# Autodesk Inventor assembly: szafka
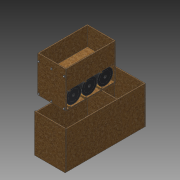
[picture p0: Inventor's stored thumbnail of the model, 180x180]
Saved by Autodesk Inventor 2013 (Build 170138000, 138)
## iProperties
Created: 2014-04-26
Part Number: szafka
Document SubType Name: Assembly
Designer: Masta
Author: Masta
## Documents named in this file (8)
- D:\prusa i3\assembly\szafka\szafka.iam
- D:\prusa i3\assembly\szafka\bok.ipt
- D:\prusa i3\assembly\szafka\tyl.ipt
- D:\prusa i3\assembly\szafka\podstawa.ipt
- D:\prusa i3\assembly\szafka\polka.ipt
- D:\prusa i3\assembly\szafka\rolka_filamentu.ipt
- D:\prusa i3\assembly\szafka\gora.ipt
- D:\prusa i3\assembly\szafka\wozek.iam
## Components (22 placed, 7 different names)
1. bok:1 — Flush:2, Flush:5, Mate:5, Flush:7, Mate:10, Flush:9, Mate:13
2. bok:2 — Flush:8, Mate:6, Mate:7
3. tyl:1 — Mate:1, Flush:2, Mate:4, Flush:6, Mate:5, Flush:7, Flush:8, Mate:6, Mate:9, Mate:11, Flush:10, Mate:14
4. podstawa:1 — Mate:4, Flush:5, Flush:6, Mate:7, Mate:12
5. polka:1 — Mate:9, Mate:10, Mate:15
6. gora:1 — Mate:11, Flush:9, Flush:10, Mate:15
7. wozek:1 [sub-assembly] — Mate:12, Mate:13, Mate:14, Tangent:1, Flush:11, Tangent:2
8. rolka_filamentu:3 — Tangent:1, Flush:11, Tangent:2
9. rolka_filamentu:4
10. rolka_filamentu:5
11. rolka_filamentu:6
12. rolka_filamentu:7
13. rolka_filamentu:8
14. rolka_filamentu:9
15. rolka_filamentu:10
16. rolka_filamentu:11
17. rolka_filamentu:12
18. rolka_filamentu:13
19. rolka_filamentu:14
20. rolka_filamentu:15
21. rolka_filamentu:16
22. rolka_filamentu:17
## Component patterns: (15 elements, first: rolka_filamentu:3)
## Relationships (22: Mate 12, Flush 8, Tangent 2)
- Mate:1: tyl:1
- Flush:2: bok:1 ↔ tyl:1
- Mate:4: tyl:1 ↔ podstawa:1
- Flush:5: bok:1 ↔ podstawa:1
- Flush:6: tyl:1 ↔ podstawa:1
- Mate:5: bok:1 ↔ tyl:1
- Flush:7: bok:1 ↔ tyl:1
- Flush:8: bok:2 ↔ tyl:1
- Mate:6: bok:2 ↔ tyl:1
- Mate:7: bok:2 ↔ podstawa:1
- Mate:9: tyl:1 ↔ polka:1
- Mate:10: bok:1 ↔ polka:1
- Mate:11: tyl:1 ↔ gora:1
- Flush:9: bok:1 ↔ gora:1
- Flush:10: tyl:1 ↔ gora:1
- Mate:12 (20 mm): podstawa:1 ↔ wozek:1
- Mate:13 (5 mm): bok:1 ↔ wozek:1
- Mate:14 (5 mm): tyl:1 ↔ wozek:1
- Mate:15 (520 mm): polka:1 ↔ gora:1
- Tangent:1: wozek:1 ↔ rolka_filamentu:3
- Flush:11 (5 mm): wozek:1 ↔ rolka_filamentu:3
- Tangent:2: wozek:1 ↔ rolka_filamentu:3
